# Autodesk Inventor assembly: ABD_Version_0.1_leftleg
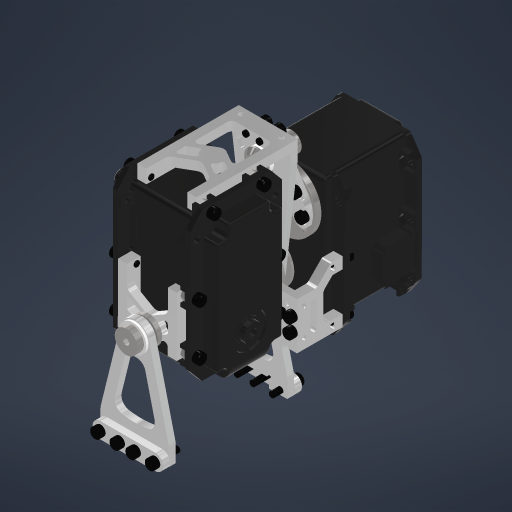
[picture p0: Inventor's stored thumbnail of the model, 512x512]
Saved by Autodesk Inventor 2024.3 (Build 283343000, 343)
## iProperties
Created: 2024-01-23
Part Number: ABD_Version_0.1_leftleg
Document SubType Name: Assembly
Designer: ASUS
Mass: 357.136 g
Surface Area: 604.848 cm^2
Volume: 181.423 cm^3
Density: 1.96853 g/cm^3
Author: ASUS
## Documents named in this file (7)
- C:\Users\ASUS\Desktop\Anti_Backlash_Structure_OP\V2_Frame(2025)\ABD_V2_Left_OP.iam
- C:\Users\ASUS\Desktop\Anti_Backlash_Structure_OP\MISUMI\Crank_Slider_Fixer.iam
- C:\Users\ASUS\Desktop\Anti_Backlash_Structure_OP\V2_Frame(2025)\Roll_Fixation_Set.iam
- C:\Users\ASUS\Desktop\Anti_Backlash_Structure_OP\V2_Frame(2025)\ABD_MX_64_Roll_Fixation_Set.iam
- C:\Users\ASUS\Desktop\Anti_Backlash_Structure_OP\V2_Frame(2025)\ABD_MX_64_Slider_Fixation_Set_Right2Horn.iam
- C:\Users\ASUS\Desktop\ABD_2024_Eindhoven\v2_Frame\ABD_Slider_Set_v2_2025.iam
- C:\Users\ASUS\Desktop\Anti_Backlash_Structure_OP\V2_Frame(2025)\MISUMI\CSH-STN-M5-6_203.ipt
## Components (6 placed, 6 different names)
1. Roll_Fixation_Set:1 [sub-assembly] — 삽입:5, 삽입:6, 각도:1, 메이트:7, 플러쉬:1
2. ABD_MX_64_Roll_Fixation_Set:1 [sub-assembly] — 메이트:2, 메이트:3, 삽입:5, 각도:1
3. ABD_MX_64_Slider_Fixation_Set_Right2Horn:1 [sub-assembly] — 메이트:2, 메이트:3, 삽입:6, 메이트:4, 메이트:6
4. Crank_Slider_Fixer:2 [sub-assembly] — 메이트:4, 메이트:6, 메이트:8
5. ABD_Slider_Set_v2_2025:1 [sub-assembly] — 메이트:7, 플러쉬:1, 메이트:8, 삽입:7
6. CSH-STN-M5-6_203:1 — 삽입:7
## Relationships (11: Mate 6, Insert 3, Angle 1, Flush 1)
- 메이트:2 [Mate] (0.05 mm): ABD_MX_64_Roll_Fixation_Set:1 ↔ ABD_MX_64_Slider_Fixation_Set_Right2Horn:1
- 메이트:3 [Mate]: ABD_MX_64_Roll_Fixation_Set:1 ↔ ABD_MX_64_Slider_Fixation_Set_Right2Horn:1
- 삽입:5 [Insert]: Roll_Fixation_Set:1 ↔ ABD_MX_64_Roll_Fixation_Set:1
- 삽입:6 [Insert]: Roll_Fixation_Set:1 ↔ ABD_MX_64_Slider_Fixation_Set_Right2Horn:1
- 각도:1 [Angle] (0 deg): Roll_Fixation_Set:1 ↔ ABD_MX_64_Roll_Fixation_Set:1
- 메이트:4 [Mate]: ABD_MX_64_Slider_Fixation_Set_Right2Horn:1 ↔ Crank_Slider_Fixer:2
- 메이트:6 [Mate]: ABD_MX_64_Slider_Fixation_Set_Right2Horn:1 ↔ Crank_Slider_Fixer:2
- 메이트:7 [Mate]: Roll_Fixation_Set:1 ↔ ABD_Slider_Set_v2_2025:1
- 플러쉬:1 [Flush] (-3 mm): Roll_Fixation_Set:1 ↔ ABD_Slider_Set_v2_2025:1
- 메이트:8 [Mate]: Crank_Slider_Fixer:2 ↔ ABD_Slider_Set_v2_2025:1
- 삽입:7 [Insert]: ABD_Slider_Set_v2_2025:1 ↔ CSH-STN-M5-6_203:1
